# Autodesk Inventor assembly: 6P 8T Sprocket, No Insert_MIR
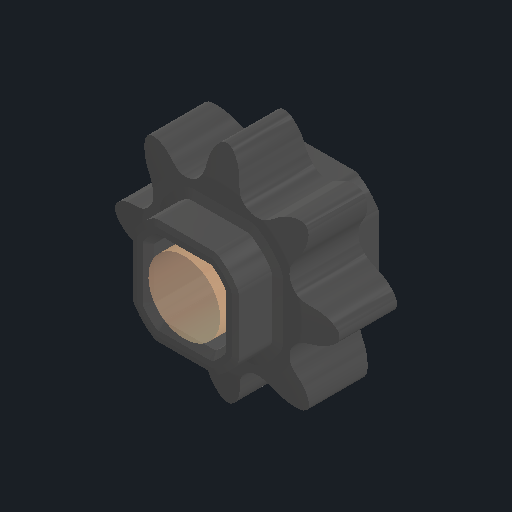
[picture p0: Inventor's stored thumbnail of the model, 512x512]
Saved by Autodesk Inventor 2026.1 (Build 301233000, 233)
## iProperties
Created: 2022-08-02
Part Number: 6P 8T Sprocket, No Insert_MIR
Document SubType Name: Assembly
Designer: roejo
Author: ylu12
## Documents named in this file (2)
- C:\Users\roejo\OneDrive\Documents\2026WorldChampionRobot\Library\VEX-CAD-Inventor-1.4.2\Motion\Sprockets\6P Sprocket\6P 8T Sprocket, No Insert_MIR.iam
- C:\Users\roejo\OneDrive\Documents\2026WorldChampionRobot\Library\VEX-CAD-Inventor-1.4.2\Motion\Sprockets\Reference Files\6P 8T Sprocket_MIR.ipt
## Components (1 placed, 1 different names)
1. 6P 8T Sprocket_MIR:1 — Flush:3, Mate:6, Mate:5
## Relationships (3: Mate 2, Flush 1)
- Flush:3: 6P 8T Sprocket_MIR:1
- Mate:6: 6P 8T Sprocket_MIR:1
- Mate:5: 6P 8T Sprocket_MIR:1
